# Autodesk Inventor assembly: OutBasePlate_InnerOutputPanel
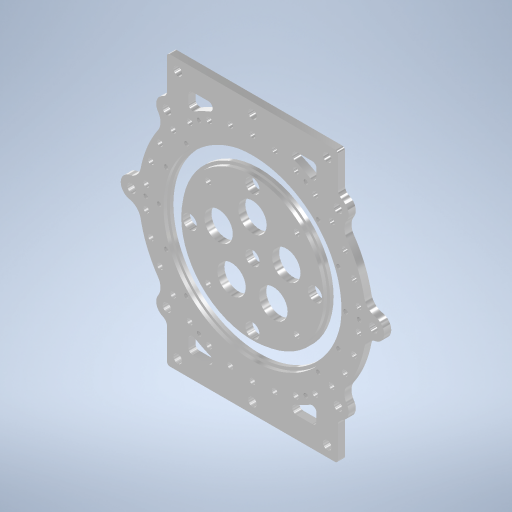
[picture p0: Inventor's stored thumbnail of the model, 512x512]
Saved by Autodesk Inventor 2024 (Build 280153000, 153)
## iProperties
Created: 2023-05-31
Part Number: OutBasePlate_InnerOutputPanel
Document SubType Name: Assembly
Designer: yuta2
Author: yuta2
## Documents named in this file (3)
- C:\Users\yuta2\Documents\Inventor\CycloidDrive\サイクロイド減速機_大型\CNC\OutBasePlate_InnerOutputPanel.iam
- C:\Users\yuta2\Documents\Inventor\CycloidDrive\サイクロイド減速機_大型\ベース板_出力側.ipt
- C:\Users\yuta2\Documents\Inventor\CycloidDrive\サイクロイド減速機_大型\出力板.ipt
## Components (2 placed, 2 different names)
1. ベース板_出力側:1 — フラッシュ:1, 挿入:1
2. 出力板:1 — フラッシュ:1, 挿入:1
## Relationships (2: Flush 1, Insert 1)
- フラッシュ:1 [Flush]: ベース板_出力側:1 ↔ 出力板:1
- 挿入:1 [Insert]: ベース板_出力側:1 ↔ 出力板:1
